# Autodesk Inventor assembly: Assembly2
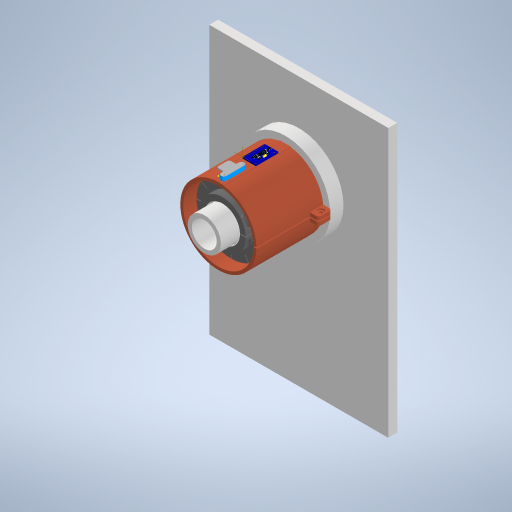
[picture p0: Inventor's stored thumbnail of the model, 512x512]
Saved by Autodesk Inventor 2023 (Build 270158000, 158)
## iProperties
Created: 2023-10-19
Part Number: Assembly2
Document SubType Name: Assembly
Designer: mark
Author: mark
## Documents named in this file (6)
- D:\Egyetem\BME MSc\Diplomamunka\opendaq\cad\EN3-01\Assembly2.iam
- D:\Egyetem\BME MSc\Diplomamunka\opendaq\cad\EN3-01\disk_12_slot.ipt
- D:\Egyetem\BME MSc\Diplomamunka\opendaq\cad\EN3-01\lathe_spindle_end.ipt
- D:\Egyetem\BME MSc\Diplomamunka\opendaq\cad\EN3-01\sensor_adapter.ipt
- D:\Egyetem\BME MSc\Diplomamunka\opendaq\cad\misc\optocoupler.ipt
- D:\Egyetem\BME MSc\Diplomamunka\opendaq\cad\misc\mpu-9250-9dof-imu-1.snapshot.4\MPU-9250.iam
## Components (5 placed, 5 different names)
1. lathe_spindle_end:1 — Mate:1, Mate:2, Mate:11
2. sensor_adapter:1 — Mate:1, Mate:2, Mate:5, Mate:6, Mate:7, Mate:8, Mate:9, Mate:10
3. optocoupler:1 — Mate:5, Mate:6, Mate:7, Mate:12
4. MPU-9250:1 [sub-assembly] — Mate:8, Mate:9, Mate:10
5. disk_12_slot:1 — Mate:11, Mate:12
## Relationships (10: Mate 10)
- Mate:1: lathe_spindle_end:1 ↔ sensor_adapter:1
- Mate:2: lathe_spindle_end:1 ↔ sensor_adapter:1
- Mate:5: sensor_adapter:1 ↔ optocoupler:1
- Mate:6: sensor_adapter:1 ↔ optocoupler:1
- Mate:7: sensor_adapter:1 ↔ optocoupler:1
- Mate:8: sensor_adapter:1 ↔ MPU-9250:1
- Mate:9: sensor_adapter:1 ↔ MPU-9250:1
- Mate:10: sensor_adapter:1 ↔ MPU-9250:1
- Mate:11: lathe_spindle_end:1 ↔ disk_12_slot:1
- Mate:12 (1.5 mm): optocoupler:1 ↔ disk_12_slot:1
